# Autodesk Inventor assembly: Battery Cart Storage Assembly
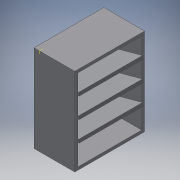
[picture p0: Inventor's stored thumbnail of the model, 180x180]
Saved by Autodesk Inventor 2018 (Build 220112000, 112)
## iProperties
Created: 2018-12-10
Part Number: Battery Cart Storage Assembly
Document SubType Name: Assembly
Designer: Gabriel
Author: Gabriel
## Documents named in this file (3)
- C:\Users\Gabriel\Documents\GitHub\2019CAD\Battery Cart Storage Assembly.iam
- C:\Users\Gabriel\Documents\Cart Box.ipt
- C:\Users\Gabriel\Documents\Cart Shelf.ipt
## Components (4 placed, 2 different names)
1. Cart Box:1 — Mate:1, Mate:2, Mate:3, Mate:4, Mate:5, Mate:6
2. Cart Shelf:1 — Mate:1, Mate:2
3. Cart Shelf:2 — Mate:5, Mate:6
4. Cart Shelf:3 — Mate:3, Mate:4
## Relationships (6: Mate 6)
- Mate:1: Cart Box:1 ↔ Cart Shelf:1
- Mate:2: Cart Box:1 ↔ Cart Shelf:1
- Mate:3: Cart Box:1 ↔ Cart Shelf:3
- Mate:4: Cart Box:1 ↔ Cart Shelf:3
- Mate:5: Cart Box:1 ↔ Cart Shelf:2
- Mate:6: Cart Box:1 ↔ Cart Shelf:2
